# Autodesk Inventor assembly: assy-shooter_base
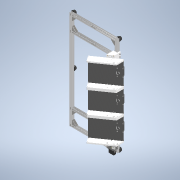
[picture p0: Inventor's stored thumbnail of the model, 180x180]
Saved by Autodesk Inventor 2022 (Build 260153000, 153)
## iProperties
Created: 2021-10-14
Part Number: assy-shooter_base
Document SubType Name: Assembly
Designer: yuto6
Author: yuto6
## Documents named in this file (8)
- C:\Users\yuto6\Documents\catchrobo_hardware\assy-shooter\assy-shooter_urdf_base.iam
- C:\Users\yuto6\Documents\catchrobo_hardware\assy-shooter\s-assy-shooter_frame.iam
- C:\Users\yuto6\Documents\catchrobo_hardware\assy-shooter\s-assy-frame-connector.iam
- C:\Users\yuto6\Documents\catchrobo_hardware\assy-shooter\shooter_base4.ipt
- C:\Users\yuto6\Documents\catchrobo_hardware\assy-shooter\shooter_base1.ipt
- C:\Users\yuto6\Documents\catchrobo_hardware\assy-shooter\shooter_carbon_plate1.ipt
- C:\Users\yuto6\Documents\catchrobo_hardware\assy-shooter\s-assy-sorter_motor.iam
- C:\Users\yuto6\Documents\catchrobo_hardware\assy-shooter\s-assy-shooter_motor2.iam
## Components (18 placed, 7 different names)
1. s-assy-shooter_frame:1 [sub-assembly] — メイト:1, メイト:2, フラッシュ:1
2. s-assy-shooter_motor2:1 [sub-assembly] — メイト:15, メイト:16, メイト:17
3. s-assy-frame-connector:1 [sub-assembly] — メイト:1, メイト:2, フラッシュ:1, メイト:3, メイト:7, メイト:8
4. s-assy-frame-connector:2 [sub-assembly] — メイト:4, メイト:5, メイト:6
5. s-assy-frame-connector:3 [sub-assembly]
6. s-assy-frame-connector:4 [sub-assembly]
7. shooter_base4:1 — メイト:3, メイト:7, メイト:8, メイト:9, メイト:11, メイト:15, メイト:16, メイト:17
8. shooter_carbon_plate1:1 — メイト:9, メイト:10, メイト:11, メイト:12, メイト:13, メイト:14
9. s-assy-sorter_motor:1 [sub-assembly] — メイト:12, メイト:13, メイト:14
10. shooter_base1:1 — メイト:4, メイト:5, メイト:6, メイト:10
11. shooter_base4:2
12. shooter_carbon_plate1:2
13. s-assy-sorter_motor:2 [sub-assembly]
14. shooter_base1:2
15. shooter_base4:3
16. shooter_carbon_plate1:3
17. s-assy-sorter_motor:3 [sub-assembly]
18. shooter_base1:3
## Component patterns: (4 elements, first: s-assy-frame-connector:1), (3 elements, first: shooter_base4:1 + shooter_carbon_plate1:1 + s-assy-sorter_motor:1 + shooter_base1:1)
## Relationships (18: Mate 17, Flush 1)
- メイト:1 [Mate]: s-assy-shooter_frame:1 ↔ s-assy-frame-connector:1
- メイト:2 [Mate]: s-assy-shooter_frame:1 ↔ s-assy-frame-connector:1
- フラッシュ:1 [Flush] (90 mm): s-assy-shooter_frame:1 ↔ s-assy-frame-connector:1
- メイト:3 [Mate]: s-assy-frame-connector:1 ↔ shooter_base4:1
- メイト:4 [Mate]: s-assy-frame-connector:2 ↔ shooter_base1:1
- メイト:5 [Mate]: s-assy-frame-connector:2 ↔ shooter_base1:1
- メイト:6 [Mate]: s-assy-frame-connector:2 ↔ shooter_base1:1
- メイト:7 [Mate]: s-assy-frame-connector:1 ↔ shooter_base4:1
- メイト:8 [Mate]: s-assy-frame-connector:1 ↔ shooter_base4:1
- メイト:9 [Mate]: shooter_base4:1 ↔ shooter_carbon_plate1:1
- メイト:10 [Mate]: shooter_carbon_plate1:1 ↔ shooter_base1:1
- メイト:11 [Mate]: shooter_base4:1 ↔ shooter_carbon_plate1:1
- メイト:12 [Mate]: shooter_carbon_plate1:1 ↔ s-assy-sorter_motor:1
- メイト:13 [Mate]: shooter_carbon_plate1:1 ↔ s-assy-sorter_motor:1
- メイト:14 [Mate]: shooter_carbon_plate1:1 ↔ s-assy-sorter_motor:1
- メイト:15 [Mate]: s-assy-shooter_motor2:1 ↔ shooter_base4:1
- メイト:16 [Mate]: s-assy-shooter_motor2:1 ↔ shooter_base4:1
- メイト:17 [Mate]: s-assy-shooter_motor2:1 ↔ shooter_base4:1
